# Autodesk Inventor assembly: wheel with drive motor floor_MIR
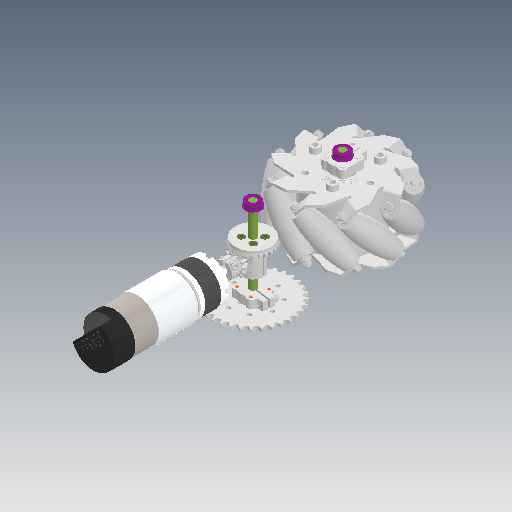
[picture p0: Inventor's stored thumbnail of the model, 512x512]
Saved by Autodesk Inventor 2020 (Build 240168000, 168)
## iProperties
Created: 2019-10-04
Part Number: wheel with drive motor floor_MIR
Document SubType Name: Assembly
Designer: ball
Author: ball
## Documents named in this file (3)
- C:\FTC\FTC8863CAD\2019 Robot\Mecanum Drive Train\wheel with drive motor floor_MIR.iam
- C:\FTC\FTC8863CAD\2019 Robot\Mecanum Drive Train\motor with bevil gear and sprocket_MIR.iam
- C:\FTC\FTC8863CAD\2019 Robot\Mecanum Drive Train\wheel with sprocket_MIR.iam
## Components (2 placed, 2 different names)
1. motor with bevil gear and sprocket_MIR:1 [sub-assembly] — Flush:5, Flush:4, Flush:3
2. wheel with sprocket_MIR:1 [sub-assembly] — Flush:5, Flush:4, Flush:3
## Relationships (3: Flush 3)
- Flush:5 (1.1684 mm): motor with bevil gear and sprocket_MIR:1 ↔ wheel with sprocket_MIR:1
- Flush:4 (-76.2 mm): motor with bevil gear and sprocket_MIR:1 ↔ wheel with sprocket_MIR:1
- Flush:3: motor with bevil gear and sprocket_MIR:1 ↔ wheel with sprocket_MIR:1
